# Autodesk Inventor assembly: BoxBeamDBAssembly
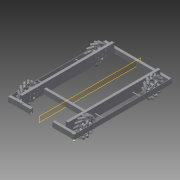
[picture p0: Inventor's stored thumbnail of the model, 180x180]
Saved by Autodesk Inventor 2015 (Build 190159000, 159)
## iProperties
Created: 2015-01-14
Part Number: BoxBeamDBAssembly
Document SubType Name: Assembly
Designer: chapale16
Author: chapale16
## Documents named in this file (15)
- \\lhssvr02\Homedirs\Robotics Club\CAD Model 2015\CDR prep\Frame\BoxBeamDBAssembly.iam
- \\lhssvr02\Homedirs\Robotics Club\CAD Model 2015\CDR prep\Frame\Frame front-back.ipt
- \\lhssvr02\Homedirs\Robotics Club\CAD Model 2015\Parts Folder\Wheels\Right Vex Mec Wheel.iam
- \\lhssvr02\Homedirs\Robotics Club\CAD Model 2015\CDR prep\Frame\Bumpers.ipt
- \\lhssvr02\Homedirs\Robotics Club\CAD Model 2015\Parts Folder\Wheels\Right Vex Mec Wheel_MIR.iam
- \\lhssvr02\Homedirs\Robotics Club\CAD Model 2015\Parts Folder\Wheels\Right Vex Mec Wheel_MIR1.iam
- \\lhssvr02\Homedirs\Robotics Club\CAD Model 2015\Parts Folder\Wheels\Right Vex Mec Wheel_MIR_MIR.iam
- \\lhssvr02\Homedirs\Robotics Club\CAD Model 2015\2x1 boxbeam 18 in.ipt
- \\lhssvr02\Homedirs\Robotics Club\CAD Model 2015\Modified Front Frame 27 in_MIR.ipt
- \\lhssvr02\Homedirs\Robotics Club\CAD Model 2015\Modified Front Frame 27 in_MIR_MIR.ipt
- \\lhssvr02\Homedirs\Robotics Club\CAD Model 2015\CDR prep\Frame\Standoffs Large.ipt
- \\lhssvr02\Homedirs\Robotics Club\CAD Model 2015\CDR prep\Frame\Standoffs Large_MIR.ipt
- \\lhssvr02\Homedirs\Robotics Club\CAD Model 2015\Box Beam Drive Base\Newest\Boxbeam.iam
- \\lhssvr02\Homedirs\Robotics Club\CAD Model 2015\Box Beam Drive Base\Newest\Boxbeam_MIR.iam
- C:\Users\whitaus15\Desktop\Random idea.ipt
## Components (17 placed, 14 different names)
1. Frame front-back:2 — Mate:6, Flush:9, Mate:7, Mate:46
2. Right Vex Mec Wheel:2 [sub-assembly] — Mate:11
3. Bumpers:1 — Mate:6, Flush:9, Mate:7, Mate:13, Flush:12, Mate:14
4. Bumpers:2 — Mate:11, Mate:43, Mate:44
5. Right Vex Mec Wheel_MIR:1 [sub-assembly]
6. Right Vex Mec Wheel_MIR1:1 [sub-assembly]
7. Right Vex Mec Wheel_MIR_MIR:1 [sub-assembly]
8. 2x1 boxbeam 18 in:1 — Mate:45
9. Modified Front Frame 27 in_MIR:2 — Mate:13, Flush:12, Mate:14, Flush:13, Mate:47, Flush:14
10. Modified Front Frame 27 in_MIR_MIR:1
11. Standoffs Large:1 — Mate:43
12. Standoffs Large:2 — Mate:44
13. Standoffs Large_MIR:1
14. Standoffs Large_MIR:2
15. Boxbeam:1 [sub-assembly] — Mate:45, Mate:46, Flush:13, Mate:48
16. Boxbeam_MIR:1 [sub-assembly]
17. Random idea:1 — Mate:47, Flush:14, Mate:48
## Relationships (15: Mate 11, Flush 4)
- Mate:6: Frame front-back:2 ↔ Bumpers:1
- Flush:9: Frame front-back:2 ↔ Bumpers:1
- Mate:7: Frame front-back:2 ↔ Bumpers:1
- Mate:11 (22.86 mm): Right Vex Mec Wheel:2 ↔ Bumpers:2
- Mate:13: Bumpers:1 ↔ Modified Front Frame 27 in_MIR:2
- Flush:12: Bumpers:1 ↔ Modified Front Frame 27 in_MIR:2
- Mate:14: Bumpers:1 ↔ Modified Front Frame 27 in_MIR:2
- Mate:43: Bumpers:2 ↔ Standoffs Large:1
- Mate:44: Bumpers:2 ↔ Standoffs Large:2
- Mate:45: 2x1 boxbeam 18 in:1 ↔ Boxbeam:1
- Mate:46: Frame front-back:2 ↔ Boxbeam:1
- Flush:13: Modified Front Frame 27 in_MIR:2 ↔ Boxbeam:1
- Mate:47: Modified Front Frame 27 in_MIR:2 ↔ Random idea:1
- Flush:14: Modified Front Frame 27 in_MIR:2 ↔ Random idea:1
- Mate:48: Boxbeam:1 ↔ Random idea:1
